# Autodesk Inventor assembly: Display
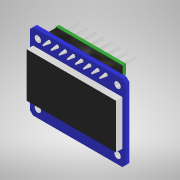
[picture p0: Inventor's stored thumbnail of the model, 180x180]
Saved by Autodesk Inventor 2022.2 (Build 262287010, 287A)
## iProperties
Created: 2026-01-01
Part Number: Display
Document SubType Name: Assembly
Designer: dbstj
Author: dbstj
## Documents named in this file (4)
- C:\Users\dbstj\Desktop\Project\5. OpenCockpit\HW\Inventor\V0.1\Display.iam
- C:\Users\dbstj\Desktop\Project\5. OpenCockpit\HW\Inventor\V0.1\SPI_Display_0.96inch.ipt
- C:\Users\dbstj\Desktop\Project\5. OpenCockpit\HW\Inventor\V0.1\board_display.ipt
- C:\Users\dbstj\Desktop\Project\5. OpenCockpit\HW\Inventor\V0.1\JST_127mm_8P.ipt
## Components (3 placed, 3 different names)
1. SPI_Display_0.96inch:1 — 메이트:1, 각도:1, 메이트:2, 메이트:3
2. board_display:1 — 메이트:1, 각도:1, 메이트:2, 메이트:3, 메이트:4, 각도:2, 메이트:5, 메이트:6
3. JST_127mm_8P:1 — 메이트:4, 각도:2, 메이트:5, 메이트:6
## Relationships (8: Mate 6, Angle 2)
- 메이트:1 [Mate]: SPI_Display_0.96inch:1 ↔ board_display:1
- 각도:1 [Angle] (0 deg): SPI_Display_0.96inch:1 ↔ board_display:1
- 메이트:2 [Mate] (-0.3 mm): SPI_Display_0.96inch:1 ↔ board_display:1
- 메이트:3 [Mate] (-0.3 mm): SPI_Display_0.96inch:1 ↔ board_display:1
- 메이트:4 [Mate]: board_display:1 ↔ JST_127mm_8P:1
- 각도:2 [Angle] (0 deg): board_display:1 ↔ JST_127mm_8P:1
- 메이트:5 [Mate] (-0.175 mm): board_display:1 ↔ JST_127mm_8P:1
- 메이트:6 [Mate] (-0.16 mm): board_display:1 ↔ JST_127mm_8P:1
